# Autodesk Inventor assembly: StrainWaveGearbox
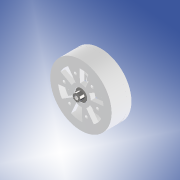
[picture p0: Inventor's stored thumbnail of the model, 180x180]
Saved by Autodesk Inventor 2017 (Build 210142000, 142)
## iProperties
Created: 2017-07-11
Part Number: StrainWaveGearbox
Document SubType Name: Assembly
Designer: zallen
Author: zallen
## Documents named in this file (11)
- C:\Users\zallen\Documents\GitHub\cr-laundry-robot\lib\Strain Wave Gearbox\StrainWaveGearbox.iam
- C:\Users\zallen\Documents\GitHub\cr-laundry-robot\lib\Strain Wave Gearbox\Flexspline.ipt
- C:\Users\zallen\Documents\GitHub\cr-laundry-robot\lib\Strain Wave Gearbox\Basespline.ipt
- C:\Users\zallen\Documents\GitHub\cr-laundry-robot\lib\Strain Wave Gearbox\WaveGenerator.ipt
- C:\Users\zallen\Documents\GitHub\cr-laundry-robot\lib\Strain Wave Gearbox\FlexsplineCover.ipt
- C:\Users\zallen\Documents\GitHub\cr-laundry-robot\lib\Strain Wave Gearbox\22x8x8mm Bearing.ipt
- C:\Users\zallen\Documents\GitHub\cr-laundry-robot\lib\Strain Wave Gearbox\WaveGeneratorRoller.ipt
- C:\Users\zallen\Documents\GitHub\cr-laundry-robot\lib\Strain Wave Gearbox\WaveGeneratorCover.ipt
- C:\Users\zallen\Documents\GitHub\cr-laundry-robot\lib\Strain Wave Gearbox\ISO 7091 - ST 8 - 100 HV.ipt
- C:\Users\zallen\Documents\GitHub\cr-laundry-robot\lib\Strain Wave Gearbox\CNS 3129 - M 8 x 1.25.ipt
- C:\Users\zallen\Documents\GitHub\cr-laundry-robot\lib\Strain Wave Gearbox\CNS 3932 - M 8 x 1.25 x 40.ipt
## Components (15 placed, 10 different names)
1. Flexspline:1 — Mate:1, Mate:6, Mate:9, Mate:10, Mate:38
2. Basespline:1 — Mate:1, Flush:2, Mate:2, Mate:3, Mate:4, Rotation:1, Mate:6, Mate:7, Flush:3, Mate:37
3. WaveGenerator:1 — Mate:4, Rotation:1, Mate:16, Mate:17, Mate:18, Mate:20, Mate:21, Mate:22, Mate:23, Mate:24, Mate:33, Rotation:2
4. FlexsplineCover:1 — Mate:9, Mate:10, Mate:11, Mate:37, Mate:38
5. 22x8x8mm Bearing:1 — Mate:7, Flush:3, Mate:32, Mate:34, Mate:35
6. 22x8x8mm Bearing:2 — Mate:11, Mate:28
7. 22x8x8mm Bearing:3 — Mate:13, Mate:16, Mate:18
8. WaveGeneratorRoller:1 — Mate:13, Mate:17
9. WaveGeneratorRoller:2 — Mate:19, Flush:4, Mate:20, Mate:21
10. 22x8x8mm Bearing:4 — Mate:19, Flush:4
11. WaveGeneratorCover:1 — Mate:22, Mate:23, Mate:24, Mate:30
12. ISO 7091 ST 8 - 100 HV:1 — Mate:30
13. CNS 3129 M 8:1 — Mate:28, Mate:36
14. ISO 7091 ST 8 - 100 HV:2 — Mate:32, Mate:33
15. CNS 3932 M 8 x 40:1 — Mate:34, Mate:35, Mate:36, Rotation:2
## Relationships (33: Mate 28, Flush 3, RelateRotation 2)
- Mate:1: Flexspline:1 ↔ Basespline:1
- Flush:2: Basespline:1
- Mate:2: Basespline:1
- Mate:3: Basespline:1
- Mate:4: Basespline:1 ↔ WaveGenerator:1
- Rotation:1 [RelateRotation] (0.0217 ul): Basespline:1 ↔ WaveGenerator:1
- Mate:6: Flexspline:1 ↔ Basespline:1
- Mate:7: Basespline:1 ↔ 22x8x8mm Bearing:1
- Flush:3: Basespline:1 ↔ 22x8x8mm Bearing:1
- Mate:9: Flexspline:1 ↔ FlexsplineCover:1
- Mate:10: Flexspline:1 ↔ FlexsplineCover:1
- Mate:11: FlexsplineCover:1 ↔ 22x8x8mm Bearing:2
- Mate:13: 22x8x8mm Bearing:3 ↔ WaveGeneratorRoller:1
- Mate:16: WaveGenerator:1 ↔ 22x8x8mm Bearing:3
- Mate:17: WaveGenerator:1 ↔ WaveGeneratorRoller:1
- Mate:18: WaveGenerator:1 ↔ 22x8x8mm Bearing:3
- Mate:19: WaveGeneratorRoller:2 ↔ 22x8x8mm Bearing:4
- Flush:4: WaveGeneratorRoller:2 ↔ 22x8x8mm Bearing:4
- Mate:20: WaveGenerator:1 ↔ WaveGeneratorRoller:2
- Mate:21: WaveGenerator:1 ↔ WaveGeneratorRoller:2
- Mate:22: WaveGenerator:1 ↔ WaveGeneratorCover:1
- Mate:23: WaveGenerator:1 ↔ WaveGeneratorCover:1
- Mate:24: WaveGenerator:1 ↔ WaveGeneratorCover:1
- Mate:28: 22x8x8mm Bearing:2 ↔ CNS 3129 M 8:1
- Mate:30: WaveGeneratorCover:1 ↔ ISO 7091 ST 8 - 100 HV:1
- Mate:32: 22x8x8mm Bearing:1 ↔ ISO 7091 ST 8 - 100 HV:2
- Mate:33: WaveGenerator:1 ↔ ISO 7091 ST 8 - 100 HV:2
- Mate:34: 22x8x8mm Bearing:1 ↔ CNS 3932 M 8 x 40:1
- Mate:35: 22x8x8mm Bearing:1 ↔ CNS 3932 M 8 x 40:1
- Mate:36: CNS 3129 M 8:1 ↔ CNS 3932 M 8 x 40:1
- Rotation:2 [RelateRotation] (1 ul): WaveGenerator:1 ↔ CNS 3932 M 8 x 40:1
- Mate:37: Basespline:1 ↔ FlexsplineCover:1
- Mate:38: Flexspline:1 ↔ FlexsplineCover:1
